# Autodesk Inventor assembly: Assembly
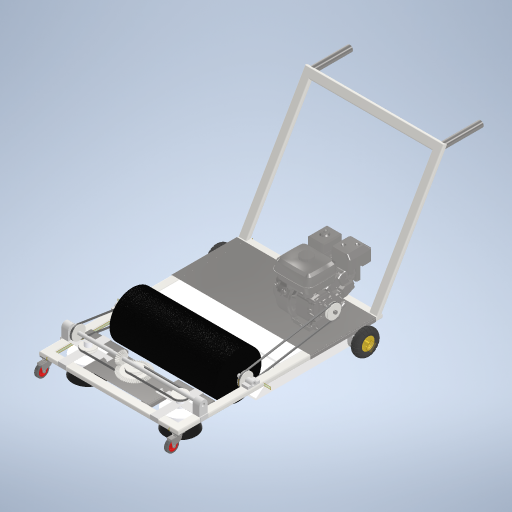
[picture p0: Inventor's stored thumbnail of the model, 512x512]
Saved by Autodesk Inventor 2024 (Build 280153000, 153)
## iProperties
_SolveAssemblyDoc: Frame Generator Solve Assembly
_Version: 15.0.0
Created: 2024-04-10
Part Number: Assembly
Document SubType Name: Assembly
Designer: teeta
Author: teeta
## Documents named in this file (27)
- C:\Users\teeta\OneDrive\Documents\Inventor\Rophi'sProject\Assembly.iam
- C:\Users\teeta\OneDrive\Documents\Inventor\Rophi'sProject\FRAME.ipt
- C:\Users\teeta\OneDrive\Documents\Inventor\Rophi'sProject\Assembly\Frame\Frame 1712736910037.iam
- C:\Users\teeta\OneDrive\Documents\Inventor\Rophi'sProject\Wheel diameter 75 mm\Wheel 75 mm Assembly.iam
- C:\Users\teeta\OneDrive\Documents\Inventor\Rophi'sProject\wheel holder.ipt
- C:\Users\teeta\OneDrive\Documents\Inventor\Rophi'sProject\10inchWheel.ipt
- C:\Users\teeta\OneDrive\Documents\Inventor\Rophi'sProject\Motor Holders.ipt
- C:\Users\teeta\OneDrive\Documents\Inventor\Rophi'sProject\GX200_Light\GX200_Light.ipt
- C:\Users\teeta\OneDrive\Documents\Inventor\Rophi'sProject\Brush_holder.ipt
- C:\Users\teeta\OneDrive\Documents\Inventor\Rophi'sProject\Brush_holder_MIR.ipt
- C:\Users\teeta\OneDrive\Documents\Inventor\Rophi'sProject\BRUSH1.ipt
- C:\Users\teeta\OneDrive\Documents\Inventor\Rophi'sProject\BRUSH1_MIR.ipt
- C:\Users\teeta\OneDrive\Documents\Inventor\Rophi'sProject\ENGINE_BASE.ipt
- C:\Users\teeta\OneDrive\Documents\Inventor\Rophi'sProject\Stand.ipt
- C:\Users\teeta\OneDrive\Documents\Inventor\Rophi'sProject\LONGI_BRUSH.ipt
- C:\Users\teeta\OneDrive\Documents\Inventor\Rophi'sProject\Assembly\Design Accelerator\V-Belt transmission1.iam
- C:\Users\teeta\OneDrive\Documents\Inventor\Rophi'sProject\BEVEL_SHAFT.ipt
- C:\Users\teeta\OneDrive\Documents\Inventor\Rophi'sProject\GEAR_SHAFT.ipt
- C:\Users\teeta\OneDrive\Documents\Inventor\Rophi'sProject\Assembly\Design Accelerator\V-Belt transmission2.iam
- C:\Users\teeta\OneDrive\Documents\Inventor\Rophi'sProject\GEAR_REST.ipt
- C:\Users\teeta\OneDrive\Documents\Inventor\Rophi'sProject\GEAR_SHAFT1.ipt
- C:\Users\teeta\OneDrive\Documents\Inventor\Rophi'sProject\Assembly\Design Accelerator\Bevel Gears1.iam
- C:\Users\teeta\OneDrive\Documents\Inventor\Rophi'sProject\Assembly\Design Accelerator\V-Belt transmission3.iam
- C:\Users\teeta\OneDrive\Documents\Inventor\Rophi'sProject\Assembly\Design Accelerator\V-Belt transmission4.iam
- C:\Users\teeta\OneDrive\Documents\Inventor\Rophi'sProject\grooves.ipt
- C:\Users\teeta\OneDrive\Documents\Inventor\Rophi'sProject\grooves_MIR.ipt
- C:\Users\teeta\OneDrive\Documents\Inventor\Rophi'sProject\DUSTPAN.ipt
## Components (29 placed, 23 different names)
1. FRAME:1 — Flush:10
2. Frame 1712736910037:1 [sub-assembly] — Mate:1, Flush:1, Flush:2, Mate:2, Flush:3, Flush:4, Flush:5, Flush:6, Mate:4, Flush:7, Flush:8, Mate:6, Flush:10, Flush:11, Flush:12, Flush:13, Flush:17, Flush:18, Mate:7, Flush:23, Flush:24, Flush:36, Flush:37, Flush:38, Flush:42, Flush:44, Flush:45, Flush:46, Flush:47
3. Wheel 75 mm Assembly:1 [sub-assembly] — Mate:2, Flush:3, Flush:4
4. Wheel 75 mm Assembly:2 [sub-assembly] — Mate:1, Flush:1, Flush:2
5. wheel holder:1 — Mate:5, Flush:8, Rotational:2, Mate:6
6. wheel holder:2 — Mate:3, Mate:4, Flush:7, Rotational:1
7. 10inchWheel:1 — Rotational:2
8. 10inchWheel:2 — Rotational:1
9. Motor Holders:1 — Flush:11
10. Brush_holder:1 — Flush:12, Flush:13
11. Brush_holder_MIR:1 — Flush:15, Flush:16, Flush:30, Flush:31
12. BRUSH1:1 — Flush:15, Flush:16
13. BRUSH1_MIR:1
14. ENGINE_BASE:1 — Flush:17, Flush:18, Flush:19, Flush:20, Flush:29
15. GX200_Light:1 — Flush:19, Flush:20, Mate:7
16. Stand:1 — Flush:23, Flush:24, Flush:25, Flush:26, Flush:27, Flush:28
17. LONGI_BRUSH:1 — Flush:25, Flush:26, Flush:27
18. V-Belt transmission:1 [sub-assembly]
19. BEVEL_SHAFT:1 — Flush:30, Flush:31, Flush:32, Flush:35, Flush:41
20. GEAR_SHAFT:1 — Flush:33, Flush:34, Flush:35, Mate:8
21. V-Belt transmission:2 [sub-assembly]
22. GEAR_REST:1 — Flush:37, Flush:38, Flush:39, Flush:40
23. GEAR_SHAFT1:1 — Flush:39, Flush:40, Mate:9
24. Bevel Gears:1 [sub-assembly] — Mate:8, Angle:1, Mate:9
25. V-Belt transmission:3 [sub-assembly]
26. V-Belt transmission:4 [sub-assembly]
27. grooves:1 — Flush:45, Flush:46
28. grooves_MIR:1
29. DUSTPAN:1
## Relationships (56: Flush 44, Mate 9, RevoluteJoint 2, Angle 1)
- Mate:1: Frame 1712736910037:1 ↔ Wheel 75 mm Assembly:2
- Flush:1: Frame 1712736910037:1 ↔ Wheel 75 mm Assembly:2
- Flush:2 (8.318 mm): Frame 1712736910037:1 ↔ Wheel 75 mm Assembly:2
- Mate:2: Frame 1712736910037:1 ↔ Wheel 75 mm Assembly:1
- Flush:3 (13.618 mm): Frame 1712736910037:1 ↔ Wheel 75 mm Assembly:1
- Flush:4: Frame 1712736910037:1 ↔ Wheel 75 mm Assembly:1
- Flush:5 (-25.4 mm): Frame 1712736910037:1
- Flush:6 (-25.4 mm): Frame 1712736910037:1
- Mate:3: wheel holder:2
- Mate:4: Frame 1712736910037:1 ↔ wheel holder:2
- Flush:7 (45 mm): Frame 1712736910037:1 ↔ wheel holder:2
- Mate:5: wheel holder:1
- Flush:8 (-45 mm): Frame 1712736910037:1 ↔ wheel holder:1
- Rotational:1 [RevoluteJoint]: wheel holder:2 ↔ 10inchWheel:2
- Rotational:2 [RevoluteJoint]: wheel holder:1 ↔ 10inchWheel:1
- Mate:6: Frame 1712736910037:1 ↔ wheel holder:1
- Flush:10 (-400 mm): FRAME:1 ↔ Frame 1712736910037:1
- Flush:11: Frame 1712736910037:1 ↔ Motor Holders:1
- Flush:12: Frame 1712736910037:1 ↔ Brush_holder:1
- Flush:13: Frame 1712736910037:1 ↔ Brush_holder:1
- Flush:14 (-187.99 mm)
- Flush:15: Brush_holder_MIR:1 ↔ BRUSH1:1
- Flush:16: Brush_holder_MIR:1 ↔ BRUSH1:1
- Flush:17: Frame 1712736910037:1 ↔ ENGINE_BASE:1
- Flush:18: Frame 1712736910037:1 ↔ ENGINE_BASE:1
- Flush:19 (120 mm): ENGINE_BASE:1 ↔ GX200_Light:1
- Flush:20 (40 mm): ENGINE_BASE:1 ↔ GX200_Light:1
- Mate:7: Frame 1712736910037:1 ↔ GX200_Light:1
- Flush:23: Frame 1712736910037:1 ↔ Stand:1
- Flush:24: Frame 1712736910037:1 ↔ Stand:1
- Flush:25: Stand:1 ↔ LONGI_BRUSH:1
- Flush:26 (-19.5 mm): Stand:1 ↔ LONGI_BRUSH:1
- Flush:27 (-19.5 mm): Stand:1 ↔ LONGI_BRUSH:1
- Flush:28 (-53 mm): Stand:1
- Flush:29 (-59.35 mm): ENGINE_BASE:1
- Flush:30: Brush_holder_MIR:1 ↔ BEVEL_SHAFT:1
- Flush:31: Brush_holder_MIR:1 ↔ BEVEL_SHAFT:1
- Flush:32 (-17.5 mm): BEVEL_SHAFT:1
- Flush:33: GEAR_SHAFT:1
- Flush:34: GEAR_SHAFT:1
- Flush:35 (-17.5 mm): BEVEL_SHAFT:1 ↔ GEAR_SHAFT:1
- Flush:36 (-77.25 mm): Frame 1712736910037:1
- Flush:37: Frame 1712736910037:1 ↔ GEAR_REST:1
- Flush:38: Frame 1712736910037:1 ↔ GEAR_REST:1
- Flush:39: GEAR_REST:1 ↔ GEAR_SHAFT1:1
- Flush:40: GEAR_REST:1 ↔ GEAR_SHAFT1:1
- Flush:41 (-422 mm): BEVEL_SHAFT:1
- Mate:8: GEAR_SHAFT:1 ↔ Bevel Gears:1
- Angle:1 (0 deg): Bevel Gears:1
- Mate:9: GEAR_SHAFT1:1 ↔ Bevel Gears:1
- Flush:42 (41.25 mm): Frame 1712736910037:1
- Flush:43 (-26.5 mm)
- Flush:44 (-708.5 mm): Frame 1712736910037:1
- Flush:45: Frame 1712736910037:1 ↔ grooves:1
- Flush:46: Frame 1712736910037:1 ↔ grooves:1
- Flush:47 (-425.4 mm): Frame 1712736910037:1
